# Autodesk Inventor assembly: frame-and-walls
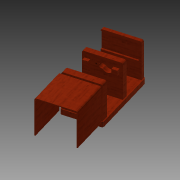
[picture p0: Inventor's stored thumbnail of the model, 180x180]
Saved by Autodesk Inventor 2015 (Build 190159000, 159)
## iProperties
Created: 2014-07-16
Part Number: frame-and-walls
Document SubType Name: Assembly
Designer: pc
Author: pc
## Documents named in this file (6)
- C:\Users\pc\Documents\blinds\openscad\frame-and-walls.iam
- C:\Users\pc\Documents\blinds\openscad\base-frame.ipt
- C:\Users\pc\Documents\blinds\openscad\wall-front.ipt
- C:\Users\pc\Documents\blinds\openscad\wall-middle.ipt
- C:\Users\pc\Documents\blinds\openscad\wall-end.ipt
- C:\Users\pc\Documents\blinds\openscad\back-cover.ipt
## Components (5 placed, 4 different names)
1. base-frame:1 — Mate:1, Mate:2, Mate:3, Mate:4, Mate:5, Mate:6, Mate:7, Mate:8, Mate:9, Mate:10
2. Front wall:1 — Mate:1, Mate:2, Mate:3, Mate:12
3. wall-middle:1 — Mate:4, Mate:5, Mate:6, Mate:11
4. wall-end:1 — Mate:7, Mate:8, Mate:9, Mate:10
5. base-frame:2 — Mate:11, Mate:12
## Relationships (12: Mate 12)
- Mate:1: base-frame:1 ↔ Front wall:1
- Mate:2: base-frame:1 ↔ Front wall:1
- Mate:3: base-frame:1 ↔ Front wall:1
- Mate:4: base-frame:1 ↔ wall-middle:1
- Mate:5: base-frame:1 ↔ wall-middle:1
- Mate:6: base-frame:1 ↔ wall-middle:1
- Mate:7: base-frame:1 ↔ wall-end:1
- Mate:8: base-frame:1 ↔ wall-end:1
- Mate:9: base-frame:1 ↔ wall-end:1
- Mate:10: base-frame:1 ↔ wall-end:1
- Mate:11: wall-middle:1 ↔ base-frame:2
- Mate:12: Front wall:1 ↔ base-frame:2
